# Autodesk Inventor assembly: Geard555
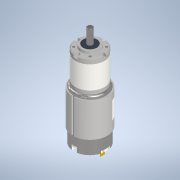
[picture p0: Inventor's stored thumbnail of the model, 180x180]
Saved by Autodesk Inventor 2022.3 (Build 263350000, 350)
## iProperties
Created: 2021-08-07
Part Number: Geard555
Document SubType Name: Assembly
Designer: Hagihara Yuya
Mass: 399 g
Surface Area: 410.721 cm^2
Volume: 40.2529 cm^3
Density: 9.91233 g/cm^3
Author: Hagihara Yuya
## Documents named in this file (3)
- C:\Users\YusukeKunita\Documents\GrabCAD\Development\BasicParts\Motor\555\Geard555.iam
- C:\Users\YusukeKunita\Documents\GrabCAD\Development\BasicParts\Motor\555\555.iam
- C:\Users\YusukeKunita\Documents\GrabCAD\Development\BasicParts\Motor\555\555_GearBox.iam
## Components (2 placed, 2 different names)
1. 555:1 [sub-assembly] — 回転:2, フラッシュ:1
2. 555_GearBox:1 [sub-assembly] — 回転:2, フラッシュ:1
## Relationships (2: RevoluteJoint 1, Flush 1)
- 回転:2 [RevoluteJoint]: 555:1 ↔ 555_GearBox:1
- フラッシュ:1 [Flush]: 555:1 ↔ 555_GearBox:1
